# Autodesk Inventor assembly: montagem.v00
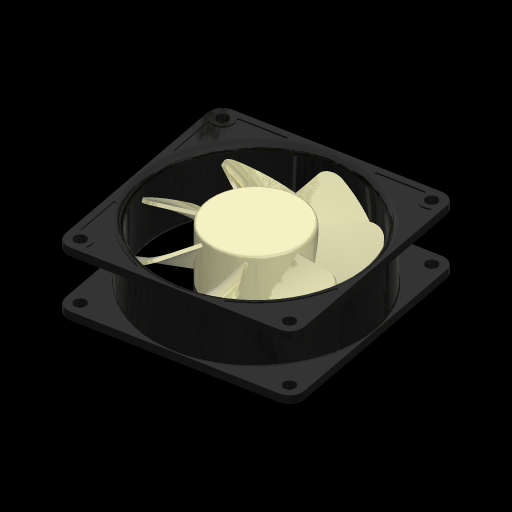
[picture p0: Inventor's stored thumbnail of the model, 512x512]
Saved by Autodesk Inventor 2023 (Build 270158000, 158)
## iProperties
Created: 2023-02-27
Part Number: montagem.v00
Document SubType Name: Assembly
Designer: @lstavares84
Author: @lstavares84
## Documents named in this file (3)
- C:\Users\tavar\OneDrive\Documentos\Inventor\cooler\montagem.v00.iam
- C:\Users\tavar\OneDrive\Documentos\Inventor\cooler\corpo.v00.ipt
- C:\Users\tavar\OneDrive\Documentos\Inventor\cooler\helice.v00.ipt
## Components (2 placed, 2 different names)
1. corpo.v00:1 — Coincidente:1, Coincidente:2, Inserir:1, Alinhado:1, Ângulo:1
2. helice.v00:1 — Inserir:1, Ângulo:1
## Relationships (5: Mate 2, Insert 1, Flush 1, Angle 1)
- Coincidente:1 [Mate]: corpo.v00:1
- Coincidente:2 [Mate]: corpo.v00:1
- Inserir:1: corpo.v00:1 ↔ helice.v00:1
- Alinhado:1 [Flush]: corpo.v00:1
- Ângulo:1 [Angle] (7200 deg): corpo.v00:1 ↔ helice.v00:1
